# Autodesk Inventor assembly: Tower Assembly
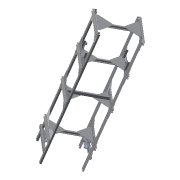
[picture p0: Inventor's stored thumbnail of the model, 180x180]
Saved by Autodesk Inventor 2015 (Build 190159000, 159)
## iProperties
Created: 2015-01-24
Part Number: Tower Assembly
Document SubType Name: Assembly
Designer: Peter
Author: Peter
## Documents named in this file (11)
- C:\Users\Tanner\Documents\GitHub\FIRST-Team-1719-CAD-Team\2015 Robot CAD\Lifter Super Structure\Tower\Tower Assembly.iam
- C:\Users\Tanner\Documents\GitHub\FIRST-Team-1719-CAD-Team\2015 Robot CAD\Lifter Super Structure\Tower\Side-Towers Assemblies\Left Side Tower Assembly.iam
- C:\Users\Tanner\Documents\GitHub\FIRST-Team-1719-CAD-Team\2015 Robot CAD\Lifter Super Structure\Tower\Side-Towers Assemblies\Right Side Tower Assembly.iam
- C:\Users\Tanner\Documents\GitHub\FIRST-Team-1719-CAD-Team\2015 Robot CAD\Lifter Super Structure\Tower\H-Shaped-Assembly\H-Shaped-Assembly.iam
- C:\Users\Tanner\Documents\GitHub\FIRST-Team-1719-CAD-Team\2015 Robot CAD\Lifter Super Structure\Tower\Side-Towers Assemblies\Right Side Tower Assembly_MIR.iam
- C:\Users\Tanner\Documents\GitHub\FIRST-Team-1719-CAD-Team\2015 Robot CAD\Lifter Super Structure\Tower\Side-Towers Assemblies\Left Side Tower Assembly_MIR.iam
- C:\Users\Tanner\Documents\GitHub\FIRST-Team-1719-CAD-Team\2015 Robot CAD\Lifter Super Structure\Tower\Elevator Motor Assembly\Elevator Motor Assembly.iam
- C:\Users\Tanner\Documents\GitHub\FIRST-Team-1719-CAD-Team\2015 Robot CAD\Lifter Super Structure\Tower\Elevator Motor Assembly\Elevator Motor Assembly_MIR1.iam
- C:\Users\Tanner\Documents\GitHub\FIRST-Team-1719-CAD-Team\2015 Robot CAD\Lifter Super Structure\Tower\Chain Tension\Chain Tension - L Bracket - Base.ipt
- C:\Users\Tanner\Documents\GitHub\FIRST-Team-1719-CAD-Team\2015 Robot CAD\Lifter Super Structure\Tower\Chain Tension\Chain Tension - L Bracket.ipt
- C:\Users\Tanner\Documents\GitHub\FIRST-Team-1719-CAD-Team\Team 1719 Parts Library\pulley  pinion 1 in 16T 615378 mod1.ipt
## Components (22 placed, 10 different names)
1. Right Side Tower Assembly:1 [sub-assembly] — Mate:1, Flush:1, Flush:2, Flush:9, Mate:5, Flush:11, Flush:12, Symmetry:1, Mate:10
2. H-Shaped-Assembly:4 [sub-assembly] — Mate:1, Flush:1, Flush:2, Flush:3, Mate:2, Flush:4
3. Left Side Tower Assembly:1 [sub-assembly] — Flush:3, Mate:2, Flush:4, Mate:3, Mate:4, Flush:5, Flush:6, Flush:7, Flush:8, Flush:10, Mate:6, Mate:8
4. H-Shaped-Assembly:5 [sub-assembly] — Mate:3, Flush:5, Flush:8, Mate:7, Flush:13, Mate:9, Flush:14, Mate:11, Mate:12, Flush:15, Flush:16
5. H-Shaped-Assembly:6 [sub-assembly] — Mate:4, Flush:6, Flush:7
6. H-Shaped-Assembly:7 [sub-assembly] — Flush:9, Mate:5, Flush:10
7. Right Side Tower Assembly_MIR:1 [sub-assembly] — Symmetry:1, Mate:15
8. Left Side Tower Assembly_MIR:1 [sub-assembly] — Mate:13, Mate:14
9. Elevator Motor Assembly:1 [sub-assembly] — Mate:6, Flush:11, Flush:12
10. Elevator Motor Assembly_MIR1:1 [sub-assembly]
11. Chain Tension - L Bracket - Base:1 — Mate:11, Mate:14, Flush:16, Insert:4
12. Chain Tension - L Bracket - Base:2 — Mate:12, Mate:13, Flush:15, Insert:3, Mate:15
13. Chain Tension - L Bracket - Base:3 — Mate:9, Flush:14, Mate:10, Insert:1
14. Chain Tension - L Bracket - Base:4 — Mate:7, Flush:13, Mate:8, Insert:2
15. Chain Tension - L Bracket:1 — Insert:1, Insert:6
16. Chain Tension - L Bracket:2 — Insert:4, Insert:8
17. Chain Tension - L Bracket:3 — Insert:2, Insert:5
18. Chain Tension - L Bracket:4 — Insert:3, Insert:7
19. pulley  pinion 1 in 16T 615378 mod1:1 — Insert:5
20. pulley  pinion 1 in 16T 615378 mod1:5 — Insert:8
21. pulley  pinion 1 in 16T 615378 mod1:6 — Insert:6
22. pulley  pinion 1 in 16T 615378 mod1:7 — Insert:7
## Relationships (40: Flush 16, Mate 15, Insert 8, Symmetry 1)
- Mate:1: Right Side Tower Assembly:1 ↔ H-Shaped-Assembly:4
- Flush:1: Right Side Tower Assembly:1 ↔ H-Shaped-Assembly:4
- Flush:2: Right Side Tower Assembly:1 ↔ H-Shaped-Assembly:4
- Flush:3: H-Shaped-Assembly:4 ↔ Left Side Tower Assembly:1
- Mate:2: H-Shaped-Assembly:4 ↔ Left Side Tower Assembly:1
- Flush:4: H-Shaped-Assembly:4 ↔ Left Side Tower Assembly:1
- Mate:3: Left Side Tower Assembly:1 ↔ H-Shaped-Assembly:5
- Mate:4: Left Side Tower Assembly:1 ↔ H-Shaped-Assembly:6
- Flush:5: Left Side Tower Assembly:1 ↔ H-Shaped-Assembly:5
- Flush:6: Left Side Tower Assembly:1 ↔ H-Shaped-Assembly:6
- Flush:7: Left Side Tower Assembly:1 ↔ H-Shaped-Assembly:6
- Flush:8 (-93.6625 mm): Left Side Tower Assembly:1 ↔ H-Shaped-Assembly:5
- Flush:9: Right Side Tower Assembly:1 ↔ H-Shaped-Assembly:7
- Mate:5: Right Side Tower Assembly:1 ↔ H-Shaped-Assembly:7
- Flush:10 (-93.6625 mm): Left Side Tower Assembly:1 ↔ H-Shaped-Assembly:7
- Mate:6: Left Side Tower Assembly:1 ↔ Elevator Motor Assembly:1
- Flush:11: Right Side Tower Assembly:1 ↔ Elevator Motor Assembly:1
- Flush:12 (-165.1 mm): Right Side Tower Assembly:1 ↔ Elevator Motor Assembly:1
- Symmetry:1: Right Side Tower Assembly:1 ↔ Right Side Tower Assembly_MIR:1
- Mate:7: H-Shaped-Assembly:5 ↔ Chain Tension - L Bracket - Base:4
- Flush:13: H-Shaped-Assembly:5 ↔ Chain Tension - L Bracket - Base:4
- Mate:8 (3.302 mm): Left Side Tower Assembly:1 ↔ Chain Tension - L Bracket - Base:4
- Mate:9: H-Shaped-Assembly:5 ↔ Chain Tension - L Bracket - Base:3
- Flush:14: H-Shaped-Assembly:5 ↔ Chain Tension - L Bracket - Base:3
- Mate:10 (3.302 mm): Right Side Tower Assembly:1 ↔ Chain Tension - L Bracket - Base:3
- Mate:11: H-Shaped-Assembly:5 ↔ Chain Tension - L Bracket - Base:1
- Mate:12: H-Shaped-Assembly:5 ↔ Chain Tension - L Bracket - Base:2
- Mate:13 (3.302 mm): Left Side Tower Assembly_MIR:1 ↔ Chain Tension - L Bracket - Base:2
- Mate:14 (3.302 mm): Left Side Tower Assembly_MIR:1 ↔ Chain Tension - L Bracket - Base:1
- Flush:15: H-Shaped-Assembly:5 ↔ Chain Tension - L Bracket - Base:2
- Flush:16: H-Shaped-Assembly:5 ↔ Chain Tension - L Bracket - Base:1
- Insert:1: Chain Tension - L Bracket - Base:3 ↔ Chain Tension - L Bracket:1
- Insert:2: Chain Tension - L Bracket - Base:4 ↔ Chain Tension - L Bracket:3
- Insert:3: Chain Tension - L Bracket - Base:2 ↔ Chain Tension - L Bracket:4
- Mate:15 (3.302 mm): Right Side Tower Assembly_MIR:1 ↔ Chain Tension - L Bracket - Base:2
- Insert:4: Chain Tension - L Bracket - Base:1 ↔ Chain Tension - L Bracket:2
- Insert:5: Chain Tension - L Bracket:3 ↔ pulley  pinion 1 in 16T 615378 mod1:1
- Insert:6: Chain Tension - L Bracket:1 ↔ pulley  pinion 1 in 16T 615378 mod1:6
- Insert:7: Chain Tension - L Bracket:4 ↔ pulley  pinion 1 in 16T 615378 mod1:7
- Insert:8: Chain Tension - L Bracket:2 ↔ pulley  pinion 1 in 16T 615378 mod1:5
## Named parameters: elevator_motor_mount_height = -165.1 mm
